# Autodesk Inventor assembly: Ch3-DiffHousingAsm
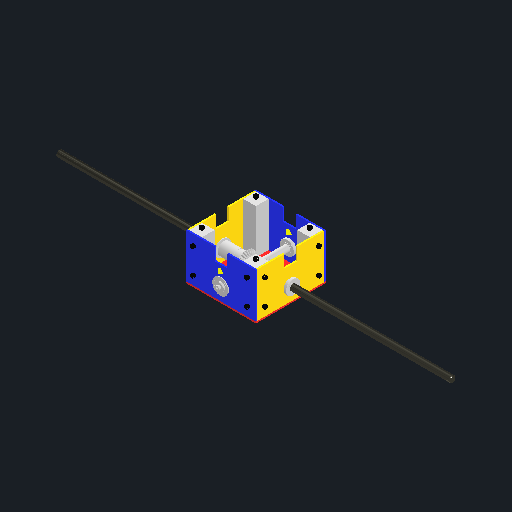
[picture p0: Inventor's stored thumbnail of the model, 512x512]
Saved by Autodesk Inventor 2026.1 (Build 301233020, 233B)
## iProperties
Created: 2023-11-30
Part Number: Ch3-DiffHousingAsm
Document SubType Name: Assembly
Designer: bugme
Author: bugme
## Documents named in this file (13)
- C:\Users\t205b\OneDrive\Documents\Github\BehrendURCMechanical\CAD\Chassis V3\Differential Box\Ch3-DiffHousingAsm.iam
- C:\Users\t205b\OneDrive\Documents\Github\BehrendURCMechanical\CAD\Chassis V3\Differential Box\DIFF_HOUSING_TOP.ipt
- C:\Users\t205b\OneDrive\Documents\Github\BehrendURCMechanical\CAD\Chassis V3\Differential Box\DIFF_PLATE_ROD.ipt
- C:\Users\t205b\OneDrive\Documents\Github\BehrendURCMechanical\CAD\Chassis V3\Differential Box\DIFF_PLATE_ROD_SHORT.ipt
- C:\Users\t205b\OneDrive\Documents\Github\BehrendURCMechanical\CAD\Chassis V3\Differential Box\1886K21_Rotary Shaft (1)\1886K21_Rotary Shaft (1).ipt
- C:\Users\t205b\OneDrive\Documents\Github\BehrendURCMechanical\CAD\Chassis V3\Differential Box\6384K361_Ball Bearing\6384K361_Ball Bearing.ipt
- C:\Users\t205b\OneDrive\Documents\Github\BehrendURCMechanical\CAD\Chassis V3\Differential Box\1886K21_Rotary Shaft (1)\1886K21_Rotary Shaft _Short.ipt
- C:\Users\t205b\OneDrive\Documents\Github\BehrendURCMechanical\CAD\Chassis V3\Differential Box\91251A342_Black-Oxide Alloy Steel Socket Head Screw\91251A342_Black-Oxide Alloy .ipt
- C:\Users\t205b\OneDrive\Documents\Github\BehrendURCMechanical\CAD\Chassis V3\Differential Box\.25 washer.ipt
- C:\Users\t205b\OneDrive\Documents\Github\BehrendURCMechanical\CAD\Chassis V3\Differential Box\CH3-DiffBoxGussetBlock.ipt
- C:\Users\t205b\OneDrive\Documents\Github\BehrendURCMechanical\CAD\Chassis V3\Differential Box\6843K12_Metal Miter Gear\6843K12_Metal Miter Gear\6843K12_Metal Miter Gear.ipt
- C:\Users\t205b\OneDrive\Documents\Github\BehrendURCMechanical\CAD\Chassis V3\Differential Box\CH3-DiffBoxSpacers.ipt
- C:\Users\t205b\OneDrive\Documents\Github\BehrendURCMechanical\CAD\Chassis V3\Differential Box\CH3-DiffHousingBottom.ipt
## Components (50 placed, 12 different names)
1. CH3-DiffHousingBottom:1 — Mate:1, Flush:2, Flush:3, Mate:2, Flush:4, Flush:5, Flush:6, Mate:6, Insert:31, Insert:32, Insert:33, Insert:34, Mate:21, Mate:30, Mate:31, Mate:32, Mate:33
2. DIFF_PLATE_ROD:1 — Mate:1, Flush:2, Flush:5, Mate:4, Insert:5, Insert:15, Insert:16, Insert:17, Insert:18, Mate:26, Mate:29
3. DIFF_PLATE_ROD:3 — Flush:3, Mate:2, Flush:4, Mate:5, Flush:7, Insert:8, Insert:23, Insert:24, Insert:25, Insert:26, Mate:23, Mate:25
4. DIFF_PLATE_ROD_SHORT:1 — Mate:4, Flush:6, Insert:19, Insert:20, Insert:21, Insert:22, Mate:21, Mate:24, Mate:27, Mate:37
5. DIFF_PLATE_ROD_SHORT:2 — Mate:5, Flush:7, Mate:6, Insert:27, Insert:28, Insert:29, Insert:30, Mate:22, Mate:28, Mate:39
6. 1886K21_Rotary Shaft (1):1 — Mate:11, Mate:34, Mate:38, Mate:42
7. 1886K21_Rotary Shaft (1):2 — Mate:14, Mate:35, Mate:40, Mate:45
8. 6384K361_Ball Bearing:1 — Mate:39, Mate:40, Mate:44
9. 6384K361_Ball Bearing:2 — Mate:37, Mate:38, Mate:41
10. 6384K361_Ball Bearing:3 — Insert:5
11. 6384K361_Ball Bearing:4 — Insert:8, Cylindrical:1, Flush:8, Insert:38
12. 1886K21_Rotary Shaft _Short:1 — Cylindrical:1, Flush:8, Mate:11, Mate:14, Insert:35, Insert:36, Mate:36
13. DIFF_HOUSING_TOP:2 — Insert:11, Insert:12, Insert:13, Insert:14
14. 91251A342_Black-Oxide Alloy :3 — Insert:11
15. 91251A342_Black-Oxide Alloy :5 — Insert:17
16. 91251A342_Black-Oxide Alloy :4 — Insert:14
17. 91251A342_Black-Oxide Alloy :6 — Insert:18
18. 91251A342_Black-Oxide Alloy :7 — Insert:13
19. 91251A342_Black-Oxide Alloy :8 — Insert:16
20. 91251A342_Black-Oxide Alloy :9 — Insert:23
21. 91251A342_Black-Oxide Alloy :10 — Insert:22
22. 91251A342_Black-Oxide Alloy :11 — Insert:15
23. 91251A342_Black-Oxide Alloy :12 — Insert:12
24. 91251A342_Black-Oxide Alloy :13 — Insert:30
25. 91251A342_Black-Oxide Alloy :14 — Insert:25
26. 91251A342_Black-Oxide Alloy :15 — Insert:26
27. 91251A342_Black-Oxide Alloy :18 — Insert:28
28. 91251A342_Black-Oxide Alloy :19 — Insert:27
29. 91251A342_Black-Oxide Alloy :20 — Insert:19
30. 91251A342_Black-Oxide Alloy :21 — Insert:20
31. 91251A342_Black-Oxide Alloy :22 — Insert:24
32. 91251A342_Black-Oxide Alloy :23 — Insert:29
33. 91251A342_Black-Oxide Alloy :24 — Insert:21
34. 91251A342_Black-Oxide Alloy :25 — Insert:32
35. 91251A342_Black-Oxide Alloy :26 — Insert:34
36. 91251A342_Black-Oxide Alloy :27 — Insert:33
37. 91251A342_Black-Oxide Alloy :28 — Insert:31
38. 91251A342_Black-Oxide Alloy :29 — Insert:36
39. 91251A342_Black-Oxide Alloy :30 — Insert:35, Insert:37
40. .25 washer:1 — Insert:37
41. .25 washer:2 — Insert:38
42. CH3-DiffBoxGussetBlock:1 — Mate:22, Mate:23, Mate:33
43. CH3-DiffBoxGussetBlock:2 — Mate:24, Mate:25, Mate:31
44. CH3-DiffBoxGussetBlock:3 — Mate:28, Mate:29, Mate:30
45. CH3-DiffBoxGussetBlock:4 — Mate:26, Mate:27, Mate:32
46. 6843K12_Metal Miter Gear:1 — Mate:36
47. 6843K12_Metal Miter Gear:2 — Mate:35, Mate:46
48. 6843K12_Metal Miter Gear:3 — Mate:34, Mate:43
49. Spacer:1 — Mate:41, Mate:42, Mate:43
50. Spacer:2 — Mate:44, Mate:45, Mate:46
## Relationships (71: Mate 33, Insert 30, Flush 7, CylindricalJoint 1)
- Mate:1: CH3-DiffHousingBottom:1 ↔ DIFF_PLATE_ROD:1
- Flush:2: CH3-DiffHousingBottom:1 ↔ DIFF_PLATE_ROD:1
- Flush:3: CH3-DiffHousingBottom:1 ↔ DIFF_PLATE_ROD:3
- Mate:2: CH3-DiffHousingBottom:1 ↔ DIFF_PLATE_ROD:3
- Flush:4: CH3-DiffHousingBottom:1 ↔ DIFF_PLATE_ROD:3
- Flush:5: CH3-DiffHousingBottom:1 ↔ DIFF_PLATE_ROD:1
- Mate:4: DIFF_PLATE_ROD:1 ↔ DIFF_PLATE_ROD_SHORT:1
- Flush:6: CH3-DiffHousingBottom:1 ↔ DIFF_PLATE_ROD_SHORT:1
- Mate:5: DIFF_PLATE_ROD:3 ↔ DIFF_PLATE_ROD_SHORT:2
- Flush:7: DIFF_PLATE_ROD:3 ↔ DIFF_PLATE_ROD_SHORT:2
- Mate:6: CH3-DiffHousingBottom:1 ↔ DIFF_PLATE_ROD_SHORT:2
- Insert:5: DIFF_PLATE_ROD:1 ↔ 6384K361_Ball Bearing:3
- Insert:8: DIFF_PLATE_ROD:3 ↔ 6384K361_Ball Bearing:4
- Cylindrical:1: 6384K361_Ball Bearing:4 ↔ 1886K21_Rotary Shaft _Short:1
- Flush:8: 6384K361_Ball Bearing:4 ↔ 1886K21_Rotary Shaft _Short:1
- Mate:11 (12.7 mm): 1886K21_Rotary Shaft (1):1 ↔ 1886K21_Rotary Shaft _Short:1
- Mate:14 (12.7 mm): 1886K21_Rotary Shaft (1):2 ↔ 1886K21_Rotary Shaft _Short:1
- Insert:11: DIFF_HOUSING_TOP:2 ↔ 91251A342_Black-Oxide Alloy :3
- Insert:12: DIFF_HOUSING_TOP:2 ↔ 91251A342_Black-Oxide Alloy :12
- Insert:13: DIFF_HOUSING_TOP:2 ↔ 91251A342_Black-Oxide Alloy :7
- Insert:14: DIFF_HOUSING_TOP:2 ↔ 91251A342_Black-Oxide Alloy :4
- Insert:15: DIFF_PLATE_ROD:1 ↔ 91251A342_Black-Oxide Alloy :11
- Insert:16: DIFF_PLATE_ROD:1 ↔ 91251A342_Black-Oxide Alloy :8
- Insert:17: DIFF_PLATE_ROD:1 ↔ 91251A342_Black-Oxide Alloy :5
- Insert:18: DIFF_PLATE_ROD:1 ↔ 91251A342_Black-Oxide Alloy :6
- Insert:19: DIFF_PLATE_ROD_SHORT:1 ↔ 91251A342_Black-Oxide Alloy :20
- Insert:20: DIFF_PLATE_ROD_SHORT:1 ↔ 91251A342_Black-Oxide Alloy :21
- Insert:21: DIFF_PLATE_ROD_SHORT:1 ↔ 91251A342_Black-Oxide Alloy :24
- Insert:22: DIFF_PLATE_ROD_SHORT:1 ↔ 91251A342_Black-Oxide Alloy :10
- Insert:23: DIFF_PLATE_ROD:3 ↔ 91251A342_Black-Oxide Alloy :9
- Insert:24: DIFF_PLATE_ROD:3 ↔ 91251A342_Black-Oxide Alloy :22
- Insert:25: DIFF_PLATE_ROD:3 ↔ 91251A342_Black-Oxide Alloy :14
- Insert:26: DIFF_PLATE_ROD:3 ↔ 91251A342_Black-Oxide Alloy :15
- Insert:27: DIFF_PLATE_ROD_SHORT:2 ↔ 91251A342_Black-Oxide Alloy :19
- Insert:28: DIFF_PLATE_ROD_SHORT:2 ↔ 91251A342_Black-Oxide Alloy :18
- Insert:29: DIFF_PLATE_ROD_SHORT:2 ↔ 91251A342_Black-Oxide Alloy :23
- Insert:30: DIFF_PLATE_ROD_SHORT:2 ↔ 91251A342_Black-Oxide Alloy :13
- Insert:31: CH3-DiffHousingBottom:1 ↔ 91251A342_Black-Oxide Alloy :28
- Insert:32: CH3-DiffHousingBottom:1 ↔ 91251A342_Black-Oxide Alloy :25
- Insert:33: CH3-DiffHousingBottom:1 ↔ 91251A342_Black-Oxide Alloy :27
- Insert:34: CH3-DiffHousingBottom:1 ↔ 91251A342_Black-Oxide Alloy :26
- Insert:35: 1886K21_Rotary Shaft _Short:1 ↔ 91251A342_Black-Oxide Alloy :30
- Insert:36: 1886K21_Rotary Shaft _Short:1 ↔ 91251A342_Black-Oxide Alloy :29
- Insert:37: 91251A342_Black-Oxide Alloy :30 ↔ .25 washer:1
- Insert:38: 6384K361_Ball Bearing:4 ↔ .25 washer:2
- Mate:21: CH3-DiffHousingBottom:1 ↔ DIFF_PLATE_ROD_SHORT:1
- Mate:22: DIFF_PLATE_ROD_SHORT:2 ↔ CH3-DiffBoxGussetBlock:1
- Mate:23: DIFF_PLATE_ROD:3 ↔ CH3-DiffBoxGussetBlock:1
- Mate:24: DIFF_PLATE_ROD_SHORT:1 ↔ CH3-DiffBoxGussetBlock:2
- Mate:25: DIFF_PLATE_ROD:3 ↔ CH3-DiffBoxGussetBlock:2
- Mate:26: DIFF_PLATE_ROD:1 ↔ CH3-DiffBoxGussetBlock:4
- Mate:27: DIFF_PLATE_ROD_SHORT:1 ↔ CH3-DiffBoxGussetBlock:4
- Mate:28: DIFF_PLATE_ROD_SHORT:2 ↔ CH3-DiffBoxGussetBlock:3
- Mate:29: DIFF_PLATE_ROD:1 ↔ CH3-DiffBoxGussetBlock:3
- Mate:30: CH3-DiffHousingBottom:1 ↔ CH3-DiffBoxGussetBlock:3
- Mate:31: CH3-DiffHousingBottom:1 ↔ CH3-DiffBoxGussetBlock:2
- Mate:32: CH3-DiffHousingBottom:1 ↔ CH3-DiffBoxGussetBlock:4
- Mate:33: CH3-DiffHousingBottom:1 ↔ CH3-DiffBoxGussetBlock:1
- Mate:34: 1886K21_Rotary Shaft (1):1 ↔ 6843K12_Metal Miter Gear:3
- Mate:35: 1886K21_Rotary Shaft (1):2 ↔ 6843K12_Metal Miter Gear:2
- Mate:36: 1886K21_Rotary Shaft _Short:1 ↔ 6843K12_Metal Miter Gear:1
- Mate:37: DIFF_PLATE_ROD_SHORT:1 ↔ 6384K361_Ball Bearing:2
- Mate:38: 1886K21_Rotary Shaft (1):1 ↔ 6384K361_Ball Bearing:2
- Mate:39: DIFF_PLATE_ROD_SHORT:2 ↔ 6384K361_Ball Bearing:1
- Mate:40: 1886K21_Rotary Shaft (1):2 ↔ 6384K361_Ball Bearing:1
- Mate:41: 6384K361_Ball Bearing:2 ↔ Spacer:1
- Mate:42: 1886K21_Rotary Shaft (1):1 ↔ Spacer:1
- Mate:43: 6843K12_Metal Miter Gear:3 ↔ Spacer:1
- Mate:44: 6384K361_Ball Bearing:1 ↔ Spacer:2
- Mate:45: 1886K21_Rotary Shaft (1):2 ↔ Spacer:2
- Mate:46: 6843K12_Metal Miter Gear:2 ↔ Spacer:2
